# Autodesk Inventor assembly: HeadSlider
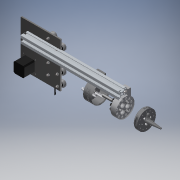
[picture p0: Inventor's stored thumbnail of the model, 180x180]
Saved by Autodesk Inventor 2017 (Build 210142000, 142)
## iProperties
Created: 2016-12-13
Part Number: HeadSlider
Document SubType Name: Assembly
Designer: umr
Mass: 1451.96 g
Surface Area: 2251.36 cm^2
Volume: 395.039 cm^3
Density: 3.67548 g/cm^3
Author: umr
## Documents named in this file (9)
- D:\SeniorProject\Models2\Head\HeadSlider.iam
- D:\SeniorProject\Models2\Head\HeadPlate.ipt
- D:\SeniorProject\Models2\Head\Solid Wheel with Eccentric Spacer Assembly.iam
- D:\SeniorProject\Models2\Head\Motor.ipt
- D:\SeniorProject\Models2\Head\GT2 20 Tooth Pulley.ipt
- D:\SeniorProject\Models2\Head\HeaderSliderBelt.ipt
- D:\SeniorProject\Models2\Head\HeaderFixer.ipt
- D:\SeniorProject\Models2\Head\M5 Screw with Tee Nut.iam
- D:\SeniorProject\Models2\UTM\UTM_Assembly.iam
## Components (20 placed, 8 different names)
1. HeadPlate:1 — Mate:3, Mate:6, Mate:8, Mate:11, Mate:18, Mate:20, Mate:21, Mate:22, Mate:23, Mate:24, Mate:42, Mate:43, Mate:44
2. Motor:1 — Mate:18, Mate:19
3. GT2 20 Tooth Pulley:1 — Mate:19, Mate:20, Mate:42
4. HeaderSliderBelt:1
5. HeaderFixer:1 — Mate:25, Mate:26, Mate:27, Mate:28, Mate:29, Mate:30, Mate:31, Mate:33, Mate:34, Mate:35, Mate:36, Mate:39
6. M5 Screw with Tee Nut:1 [sub-assembly] — Mate:21, Mate:23, Mate:25, Mate:26
7. M5 Screw with Tee Nut:2 [sub-assembly] — Mate:22, Mate:24, Mate:27
8. M5 Screw with Tee Nut:3 [sub-assembly] — Mate:28, Mate:34, Mate:40
9. M5 Screw with Tee Nut:4 [sub-assembly] — Mate:29, Mate:33, Mate:38
10. M5 Screw with Tee Nut:5 [sub-assembly] — Mate:31, Mate:36, Mate:37
11. M5 Screw with Tee Nut:6 [sub-assembly] — Mate:30, Mate:35, Mate:41
12. UTM_Assembly:1 [sub-assembly] — Mate:37, Mate:38, Mate:39, Mate:40, Mate:41
13. Solid Wheel with Eccentric Spacer Assembly:1 [sub-assembly] — Mate:3, Mate:8, Mate:43
14. Solid Wheel with Eccentric Spacer Assembly:4 [sub-assembly]
15. Solid Wheel with Eccentric Spacer Assembly:5 [sub-assembly]
16. Solid Wheel with Eccentric Spacer Assembly:6 [sub-assembly]
17. Solid Wheel with Eccentric Spacer Assembly:3 [sub-assembly] — Mate:6, Mate:11, Mate:44
18. Solid Wheel with Eccentric Spacer Assembly:7 [sub-assembly]
19. Solid Wheel with Eccentric Spacer Assembly:8 [sub-assembly]
20. Solid Wheel with Eccentric Spacer Assembly:9 [sub-assembly]
## Component patterns: (4 elements, first: Solid Wheel with Eccentric Spacer Assembly:1), (4 elements, first: Solid Wheel with Eccentric Spacer Assembly:3)
## Relationships (30: Mate 30)
- Mate:3: HeadPlate:1 ↔ Solid Wheel with Eccentric Spacer Assembly:1
- Mate:6: HeadPlate:1 ↔ Solid Wheel with Eccentric Spacer Assembly:3
- Mate:8: HeadPlate:1 ↔ Solid Wheel with Eccentric Spacer Assembly:1
- Mate:11: HeadPlate:1 ↔ Solid Wheel with Eccentric Spacer Assembly:3
- Mate:18: HeadPlate:1 ↔ Motor:1
- Mate:19: Motor:1 ↔ GT2 20 Tooth Pulley:1
- Mate:20: HeadPlate:1 ↔ GT2 20 Tooth Pulley:1
- Mate:21: HeadPlate:1 ↔ M5 Screw with Tee Nut:1
- Mate:22: HeadPlate:1 ↔ M5 Screw with Tee Nut:2
- Mate:23: HeadPlate:1 ↔ M5 Screw with Tee Nut:1
- Mate:24: HeadPlate:1 ↔ M5 Screw with Tee Nut:2
- Mate:25 (1 mm): HeaderFixer:1 ↔ M5 Screw with Tee Nut:1
- Mate:26 (3.5 mm): HeaderFixer:1 ↔ M5 Screw with Tee Nut:1
- Mate:27 (3.5 mm): HeaderFixer:1 ↔ M5 Screw with Tee Nut:2
- Mate:28 (1 mm): HeaderFixer:1 ↔ M5 Screw with Tee Nut:3
- Mate:29 (1 mm): HeaderFixer:1 ↔ M5 Screw with Tee Nut:4
- Mate:30 (1 mm): HeaderFixer:1 ↔ M5 Screw with Tee Nut:6
- Mate:31 (1 mm): HeaderFixer:1 ↔ M5 Screw with Tee Nut:5
- Mate:33 (3.5 mm): HeaderFixer:1 ↔ M5 Screw with Tee Nut:4
- Mate:34 (3.5 mm): HeaderFixer:1 ↔ M5 Screw with Tee Nut:3
- Mate:35 (3.5 mm): HeaderFixer:1 ↔ M5 Screw with Tee Nut:6
- Mate:36 (3.5 mm): HeaderFixer:1 ↔ M5 Screw with Tee Nut:5
- Mate:37: M5 Screw with Tee Nut:5 ↔ UTM_Assembly:1
- Mate:38: M5 Screw with Tee Nut:4 ↔ UTM_Assembly:1
- Mate:39: HeaderFixer:1 ↔ UTM_Assembly:1
- Mate:40: M5 Screw with Tee Nut:3 ↔ UTM_Assembly:1
- Mate:41: M5 Screw with Tee Nut:6 ↔ UTM_Assembly:1
- Mate:42: HeadPlate:1 ↔ GT2 20 Tooth Pulley:1
- Mate:43: HeadPlate:1 ↔ Solid Wheel with Eccentric Spacer Assembly:1
- Mate:44: HeadPlate:1 ↔ Solid Wheel with Eccentric Spacer Assembly:3
